# Autodesk Inventor assembly: outsideHand
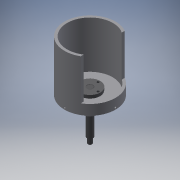
[picture p0: Inventor's stored thumbnail of the model, 180x180]
Saved by Autodesk Inventor 2016 (Build 200138000, 138)
## iProperties
Created: 2016-11-10
Part Number: outsideHand
Material: 一般
Document SubType Name: Assembly
Designer: Daisuke
Author: Daisuke
## Documents named in this file (6)
- C:\Users\Daisuke\Documents\GitHub\CAD\Hand\ver1\outsideHand.iam
- C:\Users\Daisuke\Documents\GitHub\CAD\Hand\ver1\insideBottom1.ipt
- C:\Users\Daisuke\Documents\GitHub\CAD\Hand\ver1\InsideCover.ipt
- C:\Users\Daisuke\Documents\GitHub\CAD\Hand\ver1\SSFCU12-85-F12-P8.ipt
- C:\Users\Daisuke\Documents\GitHub\CAD\Hand\ver1\STHRBN12_ss.ipt
- C:\Users\Daisuke\Documents\GitHub\CAD\Hand\ver1\Gear30.ipt
## Components (5 placed, 5 different names)
1. insideBottom1:1 — メイト:1, 挿入:1, 挿入:3, 挿入:4, 挿入:5, 挿入:6, 回転:2
2. InsideCover:1 — メイト:1, 挿入:1, 回転:3
3. SSFCU12-85-F12-P8:1 — 挿入:2, 回転:1, 回転:2, 回転:3, 回転:4
4. STHRBN12_ss:1 — 挿入:2, 挿入:3, 挿入:4, 挿入:5, 挿入:6, 回転:1, 挿入:7
5. Gear30:1 — 挿入:7, 回転:4
## Relationships (12: Insert 7, RelateRotation 4, Mate 1)
- メイト:1 [Mate]: insideBottom1:1 ↔ InsideCover:1
- 挿入:1 [Insert]: insideBottom1:1 ↔ InsideCover:1
- 挿入:2 [Insert]: SSFCU12-85-F12-P8:1 ↔ STHRBN12_ss:1
- 挿入:3 [Insert]: insideBottom1:1 ↔ STHRBN12_ss:1
- 挿入:4 [Insert]: insideBottom1:1 ↔ STHRBN12_ss:1
- 挿入:5 [Insert]: insideBottom1:1 ↔ STHRBN12_ss:1
- 挿入:6 [Insert]: insideBottom1:1 ↔ STHRBN12_ss:1
- 回転:1 [RelateRotation] (1 ul): SSFCU12-85-F12-P8:1 ↔ STHRBN12_ss:1
- 回転:2 [RelateRotation] (1 ul): insideBottom1:1 ↔ SSFCU12-85-F12-P8:1
- 回転:3 [RelateRotation] (1 ul): InsideCover:1 ↔ SSFCU12-85-F12-P8:1
- 挿入:7 [Insert]: STHRBN12_ss:1 ↔ Gear30:1
- 回転:4 [RelateRotation] (2.5 ul): SSFCU12-85-F12-P8:1 ↔ Gear30:1
